# Autodesk Inventor assembly: PCB_RT-IHU
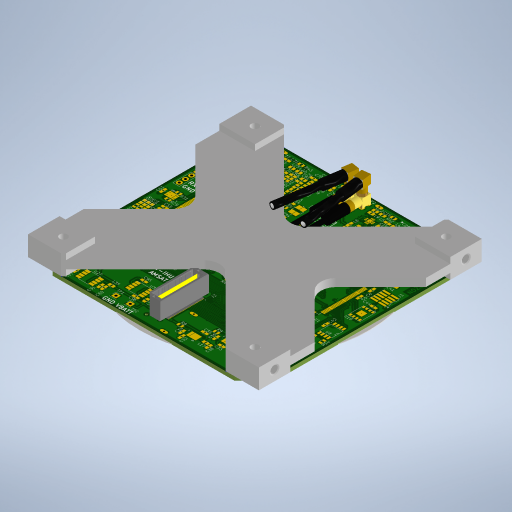
[picture p0: Inventor's stored thumbnail of the model, 512x512]
Saved by Autodesk Inventor 2023 (Build 270158000, 158)
## iProperties
Created: 2011-10-12
Part Number: PCB_RT-IHU
Document SubType Name: Assembly
Designer: Robert Davis
Description: IHU PCB
Mass: 37.4359 g
Surface Area: 203.209 cm^2
Volume: 14.8131 cm^3
Density: 2.52721 g/cm^3
Author: Robert Davis
## Documents named in this file (10)
- C:\Users\User\Downloads\CAD_backup_frequent_files_20200629 (1)\PCB_RT-IHU.iam
- C:\Users\User\Downloads\CAD_backup_frequent_files_20200629 (1)\Samtec_QSH-030-01-L-D-A.ipt
- C:\Users\User\Downloads\CAD_backup_frequent_files_20200629 (1)\Samtec_QTH-030-02-L-D-A.ipt
- C:\Users\User\Downloads\CAD_backup_frequent_files_20200629 (1)\IHU_extramass.ipt
- C:\Users\User\Downloads\CAD_backup_frequent_files_20200629 (1)\PCB_RT-IHU.ipt
- C:\Users\User\Downloads\CAD_backup_frequent_files_20200629 (1)\MMCX_thru.ipt
- C:\Users\User\Downloads\CAD_backup_frequent_files_20200629 (1)\mmcx_ra_coax_tip.ipt
- C:\Users\User\Downloads\CAD_backup_frequent_files_20200629 (1)\RT-IHU_heatsink.ipt
- C:\Users\User\Downloads\CAD_backup_frequent_files_20200629 (1)\Imported Components\MMCX-J-P-H-RA-SM1\MMCX-J-P-H-RA-SM1_body.ipt
- C:\Users\User\Downloads\CAD_backup_frequent_files_20200629 (1)\mmcx_coax_tip.ipt
## Components (13 placed, 9 different names)
1. PCB_RT-IHU:1 — Mate:3, Mate:4, Angle:3, Mate:1, Mate:2, Angle:4, Flush:1, Flush:2, Flush:3, Mate:5, Mate:11, Mate:13, Mate:14, Mate:15, Angle:5, Angle:6
2. Samtec_QTH-030-02-L-D-A:1 — Mate:1, Mate:2, Angle:4
3. Samtec_QSH-030-01-L-D-A:1 — Mate:3, Mate:4, Angle:3
4. IHU_extramass:1 — Flush:1, Flush:2, Flush:3
5. MMCX_thru:1 — Mate:5, Mate:9, Mate:10, Flush:4, Insert:2
6. MMCX_thru:2 — Mate:11, Flush:4, Mate:12, Insert:1
7. mmcx_ra_coax_tip:1 — Insert:1
8. mmcx_ra_coax_tip:2 — Insert:2
9. RT-IHU_heatsink:1 — Mate:13, Flush:5, Flush:6
10. MMCX-J-P-H-RA-SM1_body:1 — Mate:14, Angle:6, Insert:4
11. MMCX-J-P-H-RA-SM1_body:2 — Mate:15, Angle:5, Insert:3
12. mmcx_coax_tip:1 — Insert:3
13. mmcx_coax_tip:2 — Insert:4
## Relationships (26: Mate 12, Flush 6, Angle 4, Insert 4)
- Mate:3: PCB_RT-IHU:1 ↔ Samtec_QSH-030-01-L-D-A:1
- Mate:4: PCB_RT-IHU:1 ↔ Samtec_QSH-030-01-L-D-A:1
- Angle:3 (180 deg): PCB_RT-IHU:1 ↔ Samtec_QSH-030-01-L-D-A:1
- Mate:1: PCB_RT-IHU:1 ↔ Samtec_QTH-030-02-L-D-A:1
- Mate:2: PCB_RT-IHU:1 ↔ Samtec_QTH-030-02-L-D-A:1
- Angle:4 (180 deg): PCB_RT-IHU:1 ↔ Samtec_QTH-030-02-L-D-A:1
- Flush:1: PCB_RT-IHU:1 ↔ IHU_extramass:1
- Flush:2: PCB_RT-IHU:1 ↔ IHU_extramass:1
- Flush:3: PCB_RT-IHU:1 ↔ IHU_extramass:1
- Mate:5: PCB_RT-IHU:1 ↔ MMCX_thru:1
- Mate:9 (2.5 mm): MMCX_thru:1
- Mate:10 (41.75 mm): MMCX_thru:1
- Mate:11: PCB_RT-IHU:1 ↔ MMCX_thru:2
- Flush:4: MMCX_thru:1 ↔ MMCX_thru:2
- Mate:12 (-2.5 mm): MMCX_thru:2
- Insert:1: MMCX_thru:2 ↔ mmcx_ra_coax_tip:1
- Insert:2: MMCX_thru:1 ↔ mmcx_ra_coax_tip:2
- Mate:13: PCB_RT-IHU:1 ↔ RT-IHU_heatsink:1
- Flush:5: RT-IHU_heatsink:1
- Flush:6: RT-IHU_heatsink:1
- Mate:14: PCB_RT-IHU:1 ↔ MMCX-J-P-H-RA-SM1_body:1
- Mate:15: PCB_RT-IHU:1 ↔ MMCX-J-P-H-RA-SM1_body:2
- Angle:5 (0 deg): PCB_RT-IHU:1 ↔ MMCX-J-P-H-RA-SM1_body:2
- Angle:6 (0 deg): PCB_RT-IHU:1 ↔ MMCX-J-P-H-RA-SM1_body:1
- Insert:3: MMCX-J-P-H-RA-SM1_body:2 ↔ mmcx_coax_tip:1
- Insert:4: MMCX-J-P-H-RA-SM1_body:1 ↔ mmcx_coax_tip:2
